# Autodesk Inventor assembly: GE-13053
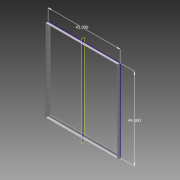
[picture p0: Inventor's stored thumbnail of the model, 180x180]
Saved by Autodesk Inventor 2013 (Build 170138000, 138)
## iProperties
Created: 2013-01-03
Part Number: GE-13053
Document SubType Name: Assembly
Designer: Phillip
_SolveAssemblyDoc: Frame Generator Solve Assembly
_Version: 15.0.0
Author: Phillip
## Documents named in this file (3)
- E:\Data Folder\FIRST 2013\FIRST KOP\FIRST Arena 2013\Feeder Goal Station\GE-13053.iam
- E:\Data Folder\FIRST 2013\FIRST KOP\FIRST Arena 2013\Feeder Goal Station\GE-13053Frame.ipt
- E:\Data Folder\FIRST 2013\FIRST KOP\FIRST Arena 2013\Feeder Goal Station\GE-13053\Frame\Frame0001.iam
## Components (2 placed, 2 different names)
1. GE-13053Frame:1
2. Frame0001:1 [sub-assembly] — Mate:1, Angle:1
## Relationships (2: Mate 1, Angle 1)
- Mate:1: Frame0001:1
- Angle:1 (0 deg): Frame0001:1
